# Autodesk Inventor assembly: turbopene
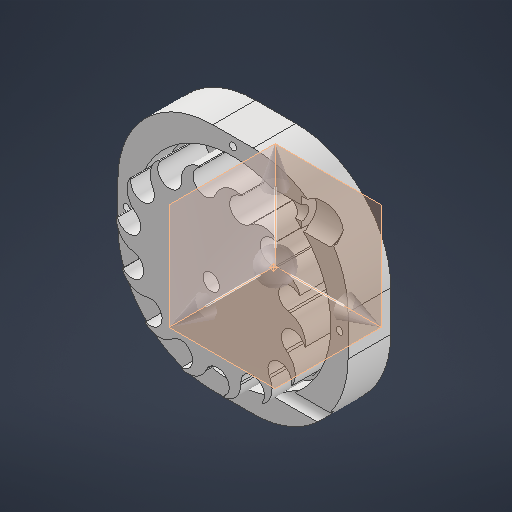
[picture p0: Inventor's stored thumbnail of the model, 512x512]
Saved by Autodesk Inventor 2025.3 (Build 293356030, 356C)
## iProperties
Created: 2025-10-02
Part Number: turbopene
Document SubType Name: Assembly
Designer: yo
Author: yo
## Documents named in this file (3)
- C:\Users\yo\Documents\Andes\9no Semestre\Proyecto Intermedio\Proyecto\Huron-Hudson\Pelton Engine\V6\Trubine_Assembly.iam
- C:\Users\yo\Documents\Andes\9no Semestre\Proyecto Intermedio\Proyecto\Huron-Hudson\Pelton Engine\V6\Turbine.ipt
- C:\Users\yo\Documents\Andes\9no Semestre\Proyecto Intermedio\Proyecto\Huron-Hudson\Pelton Engine\V6\Case.ipt
## Components (2 placed, 2 different names)
1. Case:1 — Flush:1, Flush:2, Flush:3, Mate:1, Mate:4
2. Turbine:1 — Mate:2, Mate:4
## Relationships (7: Mate 4, Flush 3)
- Flush:1: Case:1
- Flush:2: Case:1
- Flush:3: Case:1
- Mate:1: Case:1
- Mate:2: Turbine:1
- Mate:3
- Mate:4 (0.2 mm): Case:1 ↔ Turbine:1
